# Autodesk Inventor assembly: Bed Assembly
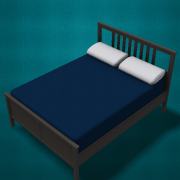
[picture p0: Inventor's stored thumbnail of the model, 180x180]
Saved by Autodesk Inventor 2017 (Build 210142000, 142)
## iProperties
Created: 2017-06-03
Part Number: Bed Assembly
Document SubType Name: Assembly
Designer: Michael
Author: Michael
## Documents named in this file (10)
- C:\Users\Michael\Google Drive\Businesses\Xatie Corp\Porfolio Pieces\Hemnes Queen Bed\Bed Assembly.iam
- C:\Users\Michael\Google Drive\Businesses\Xatie Corp\Porfolio Pieces\Hemnes Queen Bed\Header.ipt
- C:\Users\Michael\Google Drive\Businesses\Xatie Corp\Porfolio Pieces\Hemnes Queen Bed\Footer.ipt
- C:\Users\Michael\Google Drive\Businesses\Xatie Corp\Porfolio Pieces\Hemnes Queen Bed\Bed Rail.ipt
- C:\Users\Michael\Google Drive\Businesses\Xatie Corp\Porfolio Pieces\Hemnes Queen Bed\Metal Rail.ipt
- C:\Users\Michael\Google Drive\Businesses\Xatie Corp\Porfolio Pieces\Hemnes Queen Bed\Center Rail Bracket.ipt
- C:\Users\Michael\Google Drive\Businesses\Xatie Corp\Porfolio Pieces\Hemnes Queen Bed\Center Rail.ipt
- C:\Users\Michael\Google Drive\Businesses\Xatie Corp\Porfolio Pieces\Hemnes Queen Bed\Suspension Assembly.iam
- C:\Users\Michael\Google Drive\Businesses\Xatie Corp\Porfolio Pieces\Hemnes Queen Bed\Matress.ipt
- C:\Users\Michael\Google Drive\Businesses\Xatie Corp\Porfolio Pieces\Hemnes Queen Bed\Pillow.ipt
## Components (14 placed, 9 different names)
1. Header:1 — Mate:1, Mate:2, Flush:1, Flush:2, Flush:3, Mate:4, Flush:4, Flush:5, Mate:11, Angle:1
2. Footer:1 — Flush:3, Mate:3, Mate:5, Mate:6, Mate:13, Flush:15
3. Bed Rail:1 — Mate:1, Flush:1, Mate:3, Flush:5, Mate:7, Mate:8, Mate:10, Flush:10, Mate:18, Mate:20
4. Bed Rail:2 — Mate:2, Flush:2, Flush:4, Mate:9, Flush:8, Mate:17
5. Metal Rail:1 — Mate:8, Flush:6, Flush:7, Flush:9
6. Metal Rail:2 — Mate:9, Flush:6, Flush:7, Flush:8, Mate:10, Mate:19
7. Center Rail Bracket:1 — Flush:11, Mate:11, Flush:12, Mate:15
8. Center Rail:1 — Flush:9, Flush:10, Mate:15, Mate:16
9. Center Rail Bracket:2 — Flush:11, Mate:13, Mate:14
10. Suspension Assembly:1 [sub-assembly] — Flush:13, Flush:14, Mate:18
11. Suspension Assembly:2 [sub-assembly] — Flush:13, Flush:14, Mate:17, Mate:19
12. Matress:1 — Flush:15, Mate:20, Flush:16, Mate:23
13. Pillow:1 — Mate:21, Symmetry:1, Mate:22, Mate:23, Mate:24
14. Pillow:2 — Mate:21, Symmetry:1, Mate:22, Mate:24, Angle:1
## Relationships (41: Mate 23, Flush 16, Symmetry 1, Angle 1)
- Mate:1: Header:1 ↔ Bed Rail:1
- Mate:2: Header:1 ↔ Bed Rail:2
- Flush:1: Header:1 ↔ Bed Rail:1
- Flush:2: Header:1 ↔ Bed Rail:2
- Flush:3: Header:1 ↔ Footer:1
- Mate:3: Footer:1 ↔ Bed Rail:1
- Mate:4: Header:1
- Mate:5: Footer:1
- Flush:4 (12.7 mm): Header:1 ↔ Bed Rail:2
- Flush:5 (12.7 mm): Header:1 ↔ Bed Rail:1
- Mate:6: Footer:1
- Mate:7: Bed Rail:1
- Mate:8: Bed Rail:1 ↔ Metal Rail:1
- Mate:9: Bed Rail:2 ↔ Metal Rail:2
- Flush:6: Metal Rail:1 ↔ Metal Rail:2
- Flush:7: Metal Rail:1 ↔ Metal Rail:2
- Flush:8 (50.8 mm): Bed Rail:2 ↔ Metal Rail:2
- Mate:10: Bed Rail:1 ↔ Metal Rail:2
- Flush:9: Metal Rail:1 ↔ Center Rail:1
- Flush:10: Bed Rail:1 ↔ Center Rail:1
- Flush:11: Center Rail Bracket:1 ↔ Center Rail Bracket:2
- Mate:13: Footer:1 ↔ Center Rail Bracket:2
- Mate:11: Header:1 ↔ Center Rail Bracket:1
- Mate:14: Center Rail Bracket:2
- Flush:12: Center Rail Bracket:1
- Mate:15: Center Rail Bracket:1 ↔ Center Rail:1
- Mate:16: Center Rail:1
- Flush:13: Suspension Assembly:1 ↔ Suspension Assembly:2
- Flush:14: Suspension Assembly:1 ↔ Suspension Assembly:2
- Mate:17 (3.175 mm): Bed Rail:2 ↔ Suspension Assembly:2
- Mate:18 (3.175 mm): Bed Rail:1 ↔ Suspension Assembly:1
- Mate:19 (19.05 mm): Metal Rail:2 ↔ Suspension Assembly:2
- Flush:15 (-63.5 mm): Footer:1 ↔ Matress:1
- Mate:20: Bed Rail:1 ↔ Matress:1
- Flush:16: Matress:1
- Mate:21 (12.7 mm): Pillow:1 ↔ Pillow:2
- Symmetry:1: Pillow:1 ↔ Pillow:2
- Mate:22: Pillow:1 ↔ Pillow:2
- Mate:23 (71.12 mm): Matress:1 ↔ Pillow:1
- Mate:24: Pillow:1 ↔ Pillow:2
- Angle:1 (100 deg): Header:1 ↔ Pillow:2
